# Autodesk Inventor assembly: Sup_haste_sensor
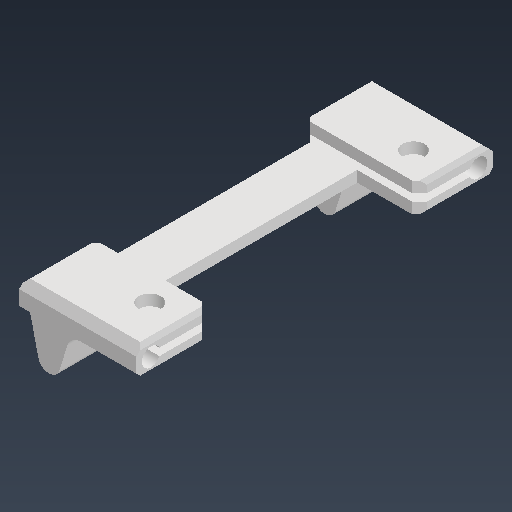
[picture p0: Inventor's stored thumbnail of the model, 512x512]
Saved by Autodesk Inventor 2026.1 (Build 301233020, 233B)
## iProperties
Created: 2026-05-08
Part Number: Sup_haste_sensor
Document SubType Name: Assembly
Designer: celio
Author: celio
## Documents named in this file (3)
- C:\Users\celio\OneDrive\Documentos\Inventor\ZeGuia\3D\Suporte\Haste sensor\Sup_haste_sensor.iam
- C:\Users\celio\OneDrive\Documentos\Inventor\ZeGuia\3D\Suporte\Haste sensor\Sup_haste_sensor_D.ipt
- C:\Users\celio\OneDrive\Documentos\Inventor\ZeGuia\3D\Suporte\Haste sensor\Sup_haste_sensor_E.ipt
## Components (2 placed, 2 different names)
1. Sup_haste_sensor_D:1 — Alinhado:1, Alinhado:2, Coincidente:1
2. Sup_haste_sensor_E:1 — Alinhado:1, Alinhado:2, Coincidente:1
## Relationships (3: Flush 2, Mate 1)
- Alinhado:1 [Flush]: Sup_haste_sensor_D:1 ↔ Sup_haste_sensor_E:1
- Alinhado:2 [Flush]: Sup_haste_sensor_D:1 ↔ Sup_haste_sensor_E:1
- Coincidente:1 [Mate] (28.646 mm): Sup_haste_sensor_D:1 ↔ Sup_haste_sensor_E:1
